# Autodesk Inventor assembly: Assembly1
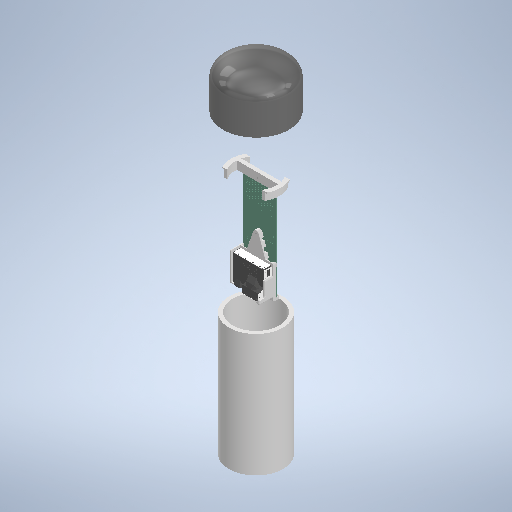
[picture p0: Inventor's stored thumbnail of the model, 512x512]
Saved by Autodesk Inventor 2025.3 (Build 293356000, 356)
## iProperties
Created: 2024-07-03
Part Number: Assembly1
Document SubType Name: Assembly
Designer: vncnt
Author: vncnt
## Documents named in this file (7)
- C:\Users\vncnt\OneDrive\Documents\Inventor\ASRC\Air Quality Sensor\Air Quality Board Mount\AQS Assembly.iam
- C:\Users\vncnt\OneDrive\Documents\Inventor\ASRC\Air Quality Sensor\Air Quality Board Mount\PVC.ipt
- C:\Users\vncnt\OneDrive\Documents\Inventor\ASRC\Air Quality Sensor\Air Quality Board Mount\CSL_AQS_V1_spin3.iam
- C:\Users\vncnt\OneDrive\Documents\Inventor\ASRC\Air Quality Sensor\Air Quality Board Mount\AQS_Mount_V5.ipt
- C:\Users\vncnt\OneDrive\Documents\Inventor\ASRC\Air Quality Sensor\Air Quality Board Mount\Sensirion_STEP_SEN5x\Sensirion_STEP_SEN5x.ipt
- C:\Users\vncnt\OneDrive\Documents\Inventor\ASRC\Air Quality Sensor\Air Quality Board Mount\3in End Cap\3in End Cap.ipt
- C:\Users\vncnt\OneDrive\Documents\Inventor\ASRC\Air Quality Sensor\Air Quality Board Mount\SEN5X_Mount_V3.ipt
## Components (6 placed, 6 different names)
1. PVC:1 — Mate:1, Mate:2, Flush:1, Mate:3, Mate:4, Mate:5, Flush:2, Mate:16
2. Sensirion_STEP_SEN5x:1 — Mate:12, Mate:13, Mate:14
3. CSL_AQS_V1_spin3:1 [sub-assembly] — Mate:5, Mate:7, Mate:9, Mate:10, Mate:11, Mate:15
4. 3in End Cap:1 — Mate:3, Mate:4
5. AQS_Mount_V5:1 — Mate:7, Flush:2, Mate:15, Mate:16
6. SEN5X_Mount_V3:1 — Mate:9, Mate:10, Mate:11, Mate:12, Mate:13, Mate:14
## Relationships (16: Mate 14, Flush 2)
- Mate:1: PVC:1
- Mate:2: PVC:1
- Flush:1: PVC:1
- Mate:3: PVC:1 ↔ 3in End Cap:1
- Mate:4: PVC:1 ↔ 3in End Cap:1
- Mate:5: PVC:1 ↔ CSL_AQS_V1_spin3:1
- Mate:7: CSL_AQS_V1_spin3:1 ↔ AQS_Mount_V5:1
- Flush:2: PVC:1 ↔ AQS_Mount_V5:1
- Mate:9: CSL_AQS_V1_spin3:1 ↔ SEN5X_Mount_V3:1
- Mate:10: CSL_AQS_V1_spin3:1 ↔ SEN5X_Mount_V3:1
- Mate:11: CSL_AQS_V1_spin3:1 ↔ SEN5X_Mount_V3:1
- Mate:12: Sensirion_STEP_SEN5x:1 ↔ SEN5X_Mount_V3:1
- Mate:13: Sensirion_STEP_SEN5x:1 ↔ SEN5X_Mount_V3:1
- Mate:14: Sensirion_STEP_SEN5x:1 ↔ SEN5X_Mount_V3:1
- Mate:15: CSL_AQS_V1_spin3:1 ↔ AQS_Mount_V5:1
- Mate:16: PVC:1 ↔ AQS_Mount_V5:1
